# Autodesk Inventor assembly: Rock Shox
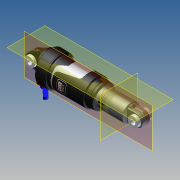
[picture p0: Inventor's stored thumbnail of the model, 180x180]
Saved by Autodesk Inventor 2014 SP2 (Build 180246200, 246)
## iProperties
Created: 2014-05-14
Part Number: Rock Shox
Document SubType Name: Assembly
Designer: Yann
Title: C:/Users/ami24/Desktop/Assemblage 1789.stp
Description: STEP AP214
Creation Date: 2013-08-27
Preprocessor: Spatial InterOp 3D
Author: Yann
## Documents named in this file (3)
- C:\Users\Yann\Documents\GitHub\PowerTrike_US\Workspaces\Espace de travail\Composants importés\Rock Shox\Rock Shox.iam
- C:\Users\Yann\Documents\GitHub\PowerTrike_US\Workspaces\Espace de travail\Composants importés\Rock Shox\Pièce 2154.ipt
- C:\Users\Yann\Documents\GitHub\PowerTrike_US\Workspaces\Espace de travail\Composants importés\Rock Shox\Pièce 2153.ipt
## Components (2 placed, 2 different names)
1. Pièce 2154 <110> — Cylindrique:1, Placage:1, Placage:2
2. Pièce 2153 <119> — Cylindrique:1, Placage:1
## Relationships (3: Mate 2, CylindricalJoint 1)
- Cylindrique:1: Pièce 2154 <110> ↔ Pièce 2153 <119>
- Placage:1 [Mate] (165 mm): Pièce 2154 <110> ↔ Pièce 2153 <119>
- Placage:2 [Mate]: Pièce 2154 <110>
